# Autodesk Inventor assembly: MotorBlock_First
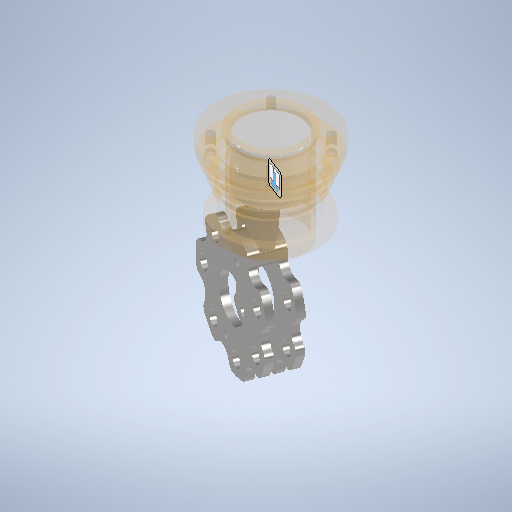
[picture p0: Inventor's stored thumbnail of the model, 512x512]
Saved by Autodesk Inventor 2025 (Build 290162010, 162A)
## iProperties
Created: 2024-07-16
Part Number: MotorBlock_First
Document SubType Name: Assembly
Designer: ffogue
Author: ffogue
## Documents named in this file (7)
- C:\Users\ffogue\OneDrive - MuM - OM\Dokumente\Inventor\Boxermotor\MotorBlock_First.iam
- C:\Users\ffogue\OneDrive - MuM - OM\Dokumente\Inventor\Boxermotor\Kolben.ipt
- C:\Users\ffogue\OneDrive - MuM - OM\Dokumente\Inventor\Boxermotor\KolbenFitting.ipt
- C:\Users\ffogue\OneDrive - MuM - OM\Dokumente\Inventor\Boxermotor\gehaeuse.ipt
- C:\Users\ffogue\OneDrive - MuM - OM\Dokumente\Inventor\Boxermotor\gehaeuse2.ipt
- C:\Users\ffogue\OneDrive - MuM - OM\Dokumente\Inventor\Boxermotor\kolbenring.ipt
- C:\Users\ffogue\OneDrive - MuM - OM\Dokumente\Inventor\Boxermotor\ring.ipt
## Components (6 placed, 6 different names)
1. gehaeuse:1 — Mate:24, Mate:26, Insert:35
2. Kolben:1 — Mate:2, Cylindrical:1, Kolbenring, Cylindrical:4, Mate:27, Flush:1
3. KolbenFitting:1 — Mate:2, Cylindrical:1, Insert:38, Flush:1
4. gehaeuse2:1 — Mate:24, Cylindrical:4, Mate:26, Mate:27, Insert:35
5. kolbenring:1 — Kolbenring
6. ring:1 — Insert:38
## Relationships (10: Mate 4, Insert 3, CylindricalJoint 2, Flush 1)
- Mate:2: Kolben:1 ↔ KolbenFitting:1
- Cylindrical:1: Kolben:1 ↔ KolbenFitting:1
- Mate:24: gehaeuse:1 ↔ gehaeuse2:1
- Kolbenring [Insert]: Kolben:1 ↔ kolbenring:1
- Cylindrical:4: Kolben:1 ↔ gehaeuse2:1
- Mate:26: gehaeuse:1 ↔ gehaeuse2:1
- Mate:27: Kolben:1 ↔ gehaeuse2:1
- Insert:35: gehaeuse:1 ↔ gehaeuse2:1
- Insert:38 (-15 mm): KolbenFitting:1 ↔ ring:1
- Flush:1: Kolben:1 ↔ KolbenFitting:1
